# Autodesk Inventor assembly: Right Leg Assembly Ver2
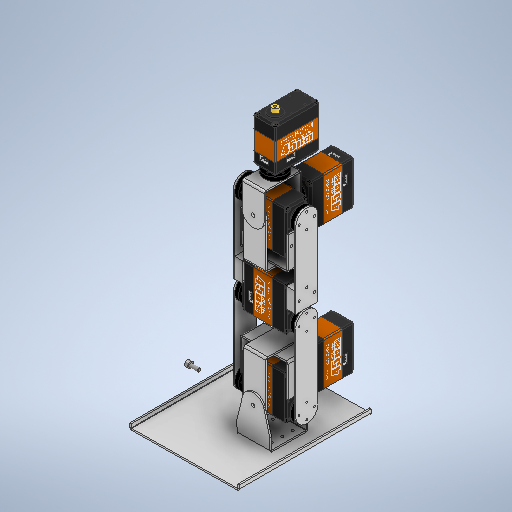
[picture p0: Inventor's stored thumbnail of the model, 512x512]
Saved by Autodesk Inventor 2025.2 (Build 292293000, 293)
## iProperties
Created: 2025-05-28
Part Number: Right Leg Assembly Ver2
Document SubType Name: Assembly
Designer: User
Author: User
## Documents named in this file (13)
- C:\Users\User\Documents\The Maverick's Files\College 3-3\로보인 프로젝트\RHp_Humanoid_ver1\Assembly\4_right_Leg.iam
- C:\Users\User\Documents\The Maverick's Files\College 3-3\로보인 프로젝트\RHp_Humanoid_ver1\Part\HTD-45H, Horn\HTD-45H\HTD-45H.iam
- C:\Users\User\Documents\The Maverick's Files\College 3-3\로보인 프로젝트\RHp_Humanoid_ver1\Part\HTD-45H, Horn\Horn\Bottom Horn.ipt
- C:\Users\User\Documents\The Maverick's Files\College 3-3\로보인 프로젝트\RHp_Humanoid_ver1\Part\Frame\Leg\axis_7_top_frame.ipt
- C:\Users\User\Documents\The Maverick's Files\College 3-3\로보인 프로젝트\RHp_Humanoid_ver1\Part\Frame\Leg\axis_9_bottom_frame.ipt
- C:\Users\User\Documents\The Maverick's Files\College 3-3\로보인 프로젝트\RHp_Humanoid_ver1\Part\HTD-45H, Horn\Horn\Top Horn.ipt
- C:\Users\User\Documents\The Maverick's Files\College 3-3\로보인 프로젝트\RHp_Humanoid_ver1\Part\Frame\Leg\axis_10_top_frame.ipt
- C:\Users\User\Documents\The Maverick's Files\College 3-3\로보인 프로젝트\RHp_Humanoid_ver1\Part\Frame\Leg\axis_8_10_connector_frame.ipt
- C:\Users\User\Documents\The Maverick's Files\College 3-3\로보인 프로젝트\RHp_Humanoid_ver1\Part\Frame\Leg\3D_printed_part.ipt
- C:\Users\User\Documents\The Maverick's Files\College 3-3\로보인 프로젝트\RHp_Humanoid_ver1\Part\Frame\Leg\axis_12_bottom_frame(bottom).ipt
- C:\Users\User\Documents\The Maverick's Files\College 3-3\로보인 프로젝트\RHp_Humanoid_ver1\Part\Frame\Leg\axis_12_bottom_frame(top).ipt
- C:\Users\User\Documents\The Maverick's Files\College 3-3\로보인 프로젝트\RHp_Humanoid_ver1\Part\Frame\Leg\axis_10_11-connector_frame.ipt
- C:\Users\User\Documents\The Maverick's Files\College 3-3\로보인 프로젝트\RHp_Humanoid_ver1\Part\Bolt, Bearing, Nut, Washer\M3x8.ipt
## Components (29 placed, 12 different names)
1. HTD-45H:1 [sub-assembly] — Flush:1, Flush:2, Mate:1, Rotational:2, Flush:3
2. HTD-45H:2 [sub-assembly] — Rotational:3, Mate:5, Mate:6, Flush:4
3. HTD-45H:3 [sub-assembly] — Rotational:4, Rotational:5, Mate:10, Mate:11, Mate:12
4. HTD-45H:4 [sub-assembly] — Mate:13, Mate:14, Flush:5, Mate:15, Rotational:6, Rotational:7
5. HTD-45H:5 [sub-assembly] — Rotational:8, Mate:19, Mate:20, Mate:21
6. HTD-45H:6 [sub-assembly] — Mate:25, Flush:12, Mate:26, Rotational:9, Rotational:11
7. Bottom Horn:1 — Rotational:2, Flush:3, Mate:2, Mate:3, Mate:4
8. Bottom Horn:2 — Rotational:5, Rigid:3
9. Bottom Horn:3 — Rotational:7, Rigid:7
10. Bottom Horn:4 — Rotational:11, Rigid:12
11. Top Horn:1 — Rotational:3, Rigid:1
12. Top Horn:2 — Rotational:4, Rigid:2
13. Top Horn:3 — Rotational:6, Rigid:11
14. Top Horn:4 — Rotational:8, Rigid:4
15. Top Horn:5 — Rotational:9, Rigid:13
16. axis_7_top_frame:1 — Mate:2, Mate:3, Mate:4, Rigid:1
17. axis_9_bottom_frame:1 — Mate:5, Mate:6, Flush:4, Mate:7, Mate:8, Mate:9
18. axis_10_top_frame:1 — Mate:7, Mate:8, Mate:9, Mate:10, Mate:11, Mate:12
19. axis_8_10_connector_frame:1 — Rigid:2, Mate:13, Mate:14, Mate:15, Mate:17, Flush:8, Flush:9
20. axis_8_10_connector_frame:2 — Rigid:3, Flush:5, Mate:16, Flush:6, Flush:7
21. 3D_printed_part:1 — Mate:16, Flush:6, Flush:7
22. 3D_printed_part:2 — Mate:17, Flush:8, Flush:9
23. axis_10_11-connector_frame:1 — Rigid:11, Rigid:13
24. axis_10_11-connector_frame:2 — Rigid:7, Rigid:12
25. axis_10_top_frame:2 — Mate:22, Mate:23, Mate:24, Mate:25, Flush:12, Mate:26
26. axis_9_bottom_frame:2 — Mate:19, Mate:20, Mate:21, Mate:22, Mate:23, Mate:24
27. axis_12_bottom_frame(top):1 — Mate:18, Flush:10, Flush:11, Rigid:4
28. axis_12_bottom_frame(bottom):1 — Mate:18, Flush:10, Flush:11
29. M3x8:1
## Relationships (55: Mate 26, Flush 12, RevoluteJoint 9, WeldJoint 8)
- Flush:1: HTD-45H:1
- Flush:2: HTD-45H:1
- Mate:1: HTD-45H:1
- Rotational:2 [RevoluteJoint]: HTD-45H:1 ↔ Bottom Horn:1
- Flush:3: HTD-45H:1 ↔ Bottom Horn:1
- Mate:2: Bottom Horn:1 ↔ axis_7_top_frame:1
- Mate:3 (2.785 mm): Bottom Horn:1 ↔ axis_7_top_frame:1
- Mate:4: Bottom Horn:1 ↔ axis_7_top_frame:1
- Rotational:3 [RevoluteJoint]: HTD-45H:2 ↔ Top Horn:1
- Mate:5: HTD-45H:2 ↔ axis_9_bottom_frame:1
- Mate:6: HTD-45H:2 ↔ axis_9_bottom_frame:1
- Flush:4 (11.5 mm): HTD-45H:2 ↔ axis_9_bottom_frame:1
- Rigid:1 [WeldJoint]: Top Horn:1 ↔ axis_7_top_frame:1
- Mate:7: axis_9_bottom_frame:1 ↔ axis_10_top_frame:1
- Mate:8: axis_9_bottom_frame:1 ↔ axis_10_top_frame:1
- Mate:9 (1.5 mm): axis_9_bottom_frame:1 ↔ axis_10_top_frame:1
- Rotational:4 [RevoluteJoint]: HTD-45H:3 ↔ Top Horn:2
- Rotational:5 [RevoluteJoint]: HTD-45H:3 ↔ Bottom Horn:2
- Mate:10: HTD-45H:3 ↔ axis_10_top_frame:1
- Mate:11: HTD-45H:3 ↔ axis_10_top_frame:1
- Mate:12 (8.5 mm): HTD-45H:3 ↔ axis_10_top_frame:1
- Rigid:2 [WeldJoint]: Top Horn:2 ↔ axis_8_10_connector_frame:1
- Rigid:3 [WeldJoint]: Bottom Horn:2 ↔ axis_8_10_connector_frame:2
- Mate:13 (7.07 mm): HTD-45H:4 ↔ axis_8_10_connector_frame:1
- Mate:14: HTD-45H:4 ↔ axis_8_10_connector_frame:1
- Flush:5: HTD-45H:4 ↔ axis_8_10_connector_frame:2
- Mate:15 (-19 mm): HTD-45H:4 ↔ axis_8_10_connector_frame:1
- Mate:16: axis_8_10_connector_frame:2 ↔ 3D_printed_part:1
- Flush:6: axis_8_10_connector_frame:2 ↔ 3D_printed_part:1
- Flush:7: axis_8_10_connector_frame:2 ↔ 3D_printed_part:1
- Mate:17: axis_8_10_connector_frame:1 ↔ 3D_printed_part:2
- Flush:8: axis_8_10_connector_frame:1 ↔ 3D_printed_part:2
- Flush:9: axis_8_10_connector_frame:1 ↔ 3D_printed_part:2
- Mate:18: axis_12_bottom_frame(top):1 ↔ axis_12_bottom_frame(bottom):1
- Flush:10: axis_12_bottom_frame(top):1 ↔ axis_12_bottom_frame(bottom):1
- Flush:11 (20 mm): axis_12_bottom_frame(top):1 ↔ axis_12_bottom_frame(bottom):1
- Rotational:6 [RevoluteJoint]: HTD-45H:4 ↔ Top Horn:3
- Rotational:7 [RevoluteJoint]: HTD-45H:4 ↔ Bottom Horn:3
- Rotational:8 [RevoluteJoint]: HTD-45H:5 ↔ Top Horn:4
- Mate:19: HTD-45H:5 ↔ axis_9_bottom_frame:2
- Mate:20: HTD-45H:5 ↔ axis_9_bottom_frame:2
- Mate:21 (-20 mm): HTD-45H:5 ↔ axis_9_bottom_frame:2
- Rigid:4 [WeldJoint]: Top Horn:4 ↔ axis_12_bottom_frame(top):1
- Mate:22: axis_10_top_frame:2 ↔ axis_9_bottom_frame:2
- Mate:23 (1.5 mm): axis_10_top_frame:2 ↔ axis_9_bottom_frame:2
- Mate:24: axis_10_top_frame:2 ↔ axis_9_bottom_frame:2
- Mate:25: HTD-45H:6 ↔ axis_10_top_frame:2
- Flush:12: HTD-45H:6 ↔ axis_10_top_frame:2
- Mate:26 (8.4 mm): HTD-45H:6 ↔ axis_10_top_frame:2
- Rotational:9 [RevoluteJoint]: HTD-45H:6 ↔ Top Horn:5
- Rigid:11 [WeldJoint]: Top Horn:3 ↔ axis_10_11-connector_frame:1
- Rotational:11 [RevoluteJoint]: HTD-45H:6 ↔ Bottom Horn:4
- Rigid:7 [WeldJoint]: Bottom Horn:3 ↔ axis_10_11-connector_frame:2
- Rigid:12 [WeldJoint]: Bottom Horn:4 ↔ axis_10_11-connector_frame:2
- Rigid:13 [WeldJoint]: Top Horn:5 ↔ axis_10_11-connector_frame:1
